# Autodesk Inventor assembly: Vert - 1in
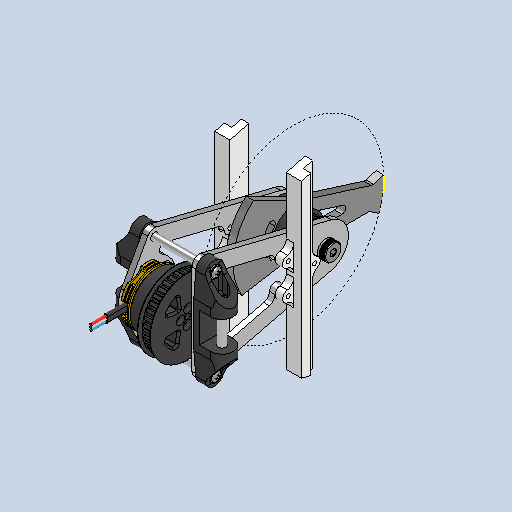
[picture p0: Inventor's stored thumbnail of the model, 512x512]
Saved by Autodesk Inventor 2023.4 (Build 274418000, 418)
## iProperties
Created: 2023-07-17
Part Number: Vert - 1in
Document SubType Name: Assembly
Designer: Nathan Cai
Mass: 662.651 g
Surface Area: 1283.02 cm^2
Volume: 224.434 cm^3
Density: 2.95254 g/cm^3
Author: Nathan Cai
## Documents named in this file (19)
- E:\Documents\Inventor\Law - V2.1\Vert - Basic\Vert - Basic.iam
- E:\Documents\Inventor\Content Center Files\R2023\en-US\ANSI B18.22.1\ANSI B18.22.1 - No. 6 - Type A.ipt
- E:\Documents\Inventor\Content Center Files\R2023\en-US\ANSI B18.6.3(27)\ANSI B18.6.3 - 6-32 UNC - 0.375(11).ipt
- E:\Documents\Inventor\Content Center Files\R2023\en-US\ANSI B18.6.3(27)\ANSI B18.6.3 - 6-32 UNC - 0.75(11).ipt
- E:\Documents\Inventor\Law - V2.1\Vert - Cheap\Needle Bearings.ipt
- E:\Documents\Inventor\Law - V2.1\Vert - Cheap\5905K497_Needle-Roller Bearing (1).ipt
- E:\Documents\Inventor\Law - V2.1\Vert - Cheap\Standoff 1.5in.ipt
- E:\Documents\Inventor\Law - V2.1\Vert - Basic\Upright - Motor.ipt
- E:\Documents\Inventor\Law - V2.1\Vert - Basic\Upright - Blank.ipt
- E:\Documents\Inventor\Law - V2.1\Vert - Basic\Leg.ipt
- E:\Documents\Inventor\Law - V2.1\Vert - Basic\FEICHAO BE4108 380KV\FEICHAO BE4108 380KV.iam
- E:\Documents\Inventor\Law - V2.1\Vert - Basic\Blade (Bar 3).ipt
- E:\Documents\Inventor\Law - V2.1\Vert - Basic\90630A121_High-Strength Steel Nylon-Insert Locknut.ipt
- E:\Documents\Inventor\Law - V2.1\Vert - Basic\XL Pulley 18T .25in Wd.ipt
- E:\Documents\Inventor\Law - V2.1\Vert - Basic\XL Pulley 36T .375in Wd.ipt
- E:\Documents\Inventor\Law - V2.1\Vert - Basic\Spacer 3-8x .125.ipt
- E:\Documents\Inventor\Law - V2.1\Vert - Basic\Standoff 1.5in.ipt
- E:\Documents\Inventor\Law - V2.1\Vert - Basic\Bracket.ipt
- E:\Documents\Inventor\Law - V2.1\Vert - Basic\91259A632_Alloy Steel Shoulder Screw\91259A632_Alloy Steel Shoulder Screw.ipt
## Components (37 placed, 17 different names)
1. FEICHAO BE4108 380KV:1 [sub-assembly] — Mate:1, Mate:11
2. Blade (Bar 3):1 — Mate:37
3. Upright - Motor:1 — Mate:1, Mate:11, Mate:24, Mate:32, Mate:103, Mate:104
4. Upright - Blank:1 — Mate:34, Mate:103, Mate:104, Mate:116, Mate:110
5. Leg:5
6. Leg:6
7. 91259A632_Alloy Steel Shoulder Screw:2
8. 90630A121_High-Strength Steel Nylon-Insert Locknut:1 — Mate:24
9. XL Pulley 18T .25in Wd:1 — Mate:37, Mate:40, Flush:2, Flush:3, Mate:107
10. XL Pulley 36T .375in Wd:1 — Flush:3
11. Spacer 3-8x .125:1 — Mate:107
12. Needle Bearings:3 — Mate:32
13. Needle Bearings:4 — Mate:34
14. 5905K497_Needle-Roller Bearing (1):3
15. 5905K497_Needle-Roller Bearing (1):4 — Mate:40, Flush:2
16. Standoff 1.5in:5 — Mate:116
17. Standoff 1.5in:6 — Mate:110
18. Cross Recessed Truss Head Machine Screw - Type I - Inch No. 6 - 32 - 3/4:5 — Insert:10
19. Plain Washer (Inch) No. 6 - Type A:8 — Mate:114, Mate:115, Insert:10
20. Cross Recessed Truss Head Machine Screw - Type I - Inch No. 6 - 32 - 3/4:1 — Insert:9
21. Plain Washer (Inch) No. 6 - Type A:7 — Mate:112, Mate:113, Insert:9
22. Bracket:1 — Mate:112, Mate:113, Mate:114, Mate:115
23. Standoff 1.5in:4
24. Plain Washer (Inch) No. 6 - Type A:1 — Insert:1
25. Cross Recessed Truss Head Machine Screw - Type I - Inch No. 6 - 32 - 3/8:1 — Insert:1
26. Plain Washer (Inch) No. 6 - Type A:2 — Insert:2
27. Cross Recessed Truss Head Machine Screw - Type I - Inch No. 6 - 32 - 3/8:2 — Insert:2
28. Standoff 1.5in:3
29. Bracket:2
30. Plain Washer (Inch) No. 6 - Type A:3 — Insert:5
31. Cross Recessed Truss Head Machine Screw - Type I - Inch No. 6 - 32 - 3/8:3 — Insert:5
32. Plain Washer (Inch) No. 6 - Type A:4 — Insert:6
33. Cross Recessed Truss Head Machine Screw - Type I - Inch No. 6 - 32 - 3/8:4 — Insert:6
34. Plain Washer (Inch) No. 6 - Type A:5 — Insert:7
35. Cross Recessed Truss Head Machine Screw - Type I - Inch No. 6 - 32 - 3/4:3 — Insert:7
36. Plain Washer (Inch) No. 6 - Type A:6 — Insert:8
37. Cross Recessed Truss Head Machine Screw - Type I - Inch No. 6 - 32 - 3/4:4 — Insert:8
## Relationships (73: Mate 59, Insert 8, Flush 6)
- Mate:1: FEICHAO BE4108 380KV:1 ↔ Upright - Motor:1
- [Mate]: FEICHAO BE4108 380KV:1 ↔ Upright - Motor:1
- [Mate]: Blade (Bar 3):1 ↔ Upright - Motor:1
- Mate:11: FEICHAO BE4108 380KV:1 ↔ Upright - Motor:1
- [Mate]: Upright - Motor:1 ↔ Leg:5
- [Mate]: Upright - Motor:1 ↔ Leg:5
- [Mate]: Upright - Motor:1 ↔ Leg:5
- [Mate]: Upright - Blank:1 ↔ Leg:6
- [Mate]: Upright - Blank:1 ↔ Leg:6
- [Mate]: Upright - Blank:1 ↔ Leg:6
- [Mate]: Upright - Blank:1 ↔ 91259A632_Alloy Steel Shoulder Screw:2
- [Mate]: Upright - Blank:1 ↔ 91259A632_Alloy Steel Shoulder Screw:2
- Mate:24: Upright - Motor:1 ↔ 90630A121_High-Strength Steel Nylon-Insert Locknut:1
- [Mate]: 91259A632_Alloy Steel Shoulder Screw:2 ↔ 90630A121_High-Strength Steel Nylon-Insert Locknut:1
- [Mate]: Blade (Bar 3):1 ↔ Spacer 3-8x .125:1
- [Mate]: Blade (Bar 3):1 ↔ Spacer 3-8x .125:1
- [Mate]: 91259A632_Alloy Steel Shoulder Screw:2 ↔ Needle Bearings:3
- Mate:32: Upright - Motor:1 ↔ Needle Bearings:3
- [Mate]: 91259A632_Alloy Steel Shoulder Screw:2 ↔ Needle Bearings:4
- Mate:34: Upright - Blank:1 ↔ Needle Bearings:4
- Mate:37: Blade (Bar 3):1 ↔ XL Pulley 18T .25in Wd:1
- [Mate]: Blade (Bar 3):1 ↔ Spacer 3-8x .125:1
- Mate:40: XL Pulley 18T .25in Wd:1 ↔ 5905K497_Needle-Roller Bearing (1):4
- [Mate]: Blade (Bar 3):1 ↔ 5905K497_Needle-Roller Bearing (1):3
- [Flush]: Spacer 3-8x .125:1 ↔ 5905K497_Needle-Roller Bearing (1):3
- Flush:2: XL Pulley 18T .25in Wd:1 ↔ 5905K497_Needle-Roller Bearing (1):4
- [Mate]: Spacer 3-8x .125:1 ↔ Needle Bearings:3
- Flush:3: XL Pulley 18T .25in Wd:1 ↔ XL Pulley 36T .375in Wd:1
- [Mate]: FEICHAO BE4108 380KV:1 ↔ XL Pulley 36T .375in Wd:1
- [Mate]: FEICHAO BE4108 380KV:1 ↔ XL Pulley 36T .375in Wd:1
- [Mate]: Upright - Motor:1 ↔ Bracket:1
- [Mate]: Upright - Motor:1 ↔ Bracket:1
- [Mate]: Bracket:1 ↔ Standoff 1.5in:4
- [Flush]: Bracket:1 ↔ Standoff 1.5in:4
- [Mate]: Standoff 1.5in:4 ↔ Plain Washer (Inch) No. 6 - Type A:1
- [Mate]: Standoff 1.5in:4 ↔ Plain Washer (Inch) No. 6 - Type A:1
- Insert:1: Plain Washer (Inch) No. 6 - Type A:1 ↔ Cross Recessed Truss Head Machine Screw - Type I - Inch No. 6 - 32 - 3/8:1
- [Mate]: Standoff 1.5in:4 ↔ Plain Washer (Inch) No. 6 - Type A:2
- [Mate]: Standoff 1.5in:4 ↔ Plain Washer (Inch) No. 6 - Type A:2
- Insert:2: Plain Washer (Inch) No. 6 - Type A:2 ↔ Cross Recessed Truss Head Machine Screw - Type I - Inch No. 6 - 32 - 3/8:2
- [Mate]: Standoff 1.5in:3 ↔ Bracket:2
- [Flush]: Standoff 1.5in:3 ↔ Bracket:2
- [Mate]: Standoff 1.5in:3 ↔ Plain Washer (Inch) No. 6 - Type A:3
- [Mate]: Standoff 1.5in:3 ↔ Plain Washer (Inch) No. 6 - Type A:3
- Insert:5: Plain Washer (Inch) No. 6 - Type A:3 ↔ Cross Recessed Truss Head Machine Screw - Type I - Inch No. 6 - 32 - 3/8:3
- [Mate]: Standoff 1.5in:3 ↔ Plain Washer (Inch) No. 6 - Type A:4
- [Mate]: Standoff 1.5in:3 ↔ Plain Washer (Inch) No. 6 - Type A:4
- Insert:6: Plain Washer (Inch) No. 6 - Type A:4 ↔ Cross Recessed Truss Head Machine Screw - Type I - Inch No. 6 - 32 - 3/8:4
- [Mate]: Bracket:2 ↔ Plain Washer (Inch) No. 6 - Type A:5
- [Mate]: Bracket:2 ↔ Plain Washer (Inch) No. 6 - Type A:5
- [Mate]: Bracket:2 ↔ Plain Washer (Inch) No. 6 - Type A:6
- [Mate]: Bracket:2 ↔ Plain Washer (Inch) No. 6 - Type A:6
- Insert:7: Plain Washer (Inch) No. 6 - Type A:5 ↔ Cross Recessed Truss Head Machine Screw - Type I - Inch No. 6 - 32 - 3/4:3
- Insert:8: Plain Washer (Inch) No. 6 - Type A:6 ↔ Cross Recessed Truss Head Machine Screw - Type I - Inch No. 6 - 32 - 3/4:4
- [Flush]: Bracket:1 ↔ Bracket:2
- [Mate]: Bracket:1 ↔ Bracket:2
- [Mate]: Upright - Blank:1 ↔ Bracket:2
- [Mate]: Upright - Motor:1 ↔ Bracket:1
- Mate:103: Upright - Motor:1 ↔ Upright - Blank:1
- Mate:104 (38.1 mm): Upright - Motor:1 ↔ Upright - Blank:1
- [Mate]: 91259A632_Alloy Steel Shoulder Screw:2 ↔ XL Pulley 18T .25in Wd:1
- [Mate]: Upright - Motor:1 ↔ 91259A632_Alloy Steel Shoulder Screw:2
- Mate:107: XL Pulley 18T .25in Wd:1 ↔ Spacer 3-8x .125:1
- [Mate]: Upright - Motor:1 ↔ Standoff 1.5in:5
- Mate:110: Upright - Blank:1 ↔ Standoff 1.5in:6
- [Mate]: Upright - Motor:1 ↔ Standoff 1.5in:6
- Mate:112: Plain Washer (Inch) No. 6 - Type A:7 ↔ Bracket:1
- Mate:113: Plain Washer (Inch) No. 6 - Type A:7 ↔ Bracket:1
- Mate:114: Plain Washer (Inch) No. 6 - Type A:8 ↔ Bracket:1
- Mate:115: Plain Washer (Inch) No. 6 - Type A:8 ↔ Bracket:1
- Insert:9: Cross Recessed Truss Head Machine Screw - Type I - Inch No. 6 - 32 - 3/4:1 ↔ Plain Washer (Inch) No. 6 - Type A:7
- Insert:10: Cross Recessed Truss Head Machine Screw - Type I - Inch No. 6 - 32 - 3/4:5 ↔ Plain Washer (Inch) No. 6 - Type A:8
- Mate:116: Upright - Blank:1 ↔ Standoff 1.5in:5
